# Autodesk Inventor assembly: slide with inserts
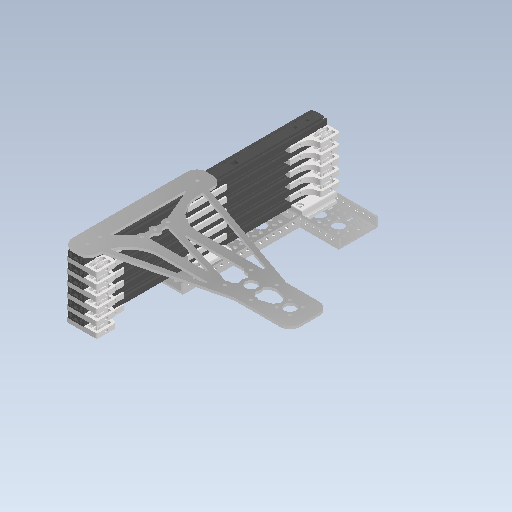
[picture p0: Inventor's stored thumbnail of the model, 512x512]
Saved by Autodesk Inventor 2020 (Build 240168000, 168)
## iProperties
Created: 2019-12-18
Part Number: slide with inserts
Document SubType Name: Assembly
Designer: xj82b
Author: xj82b
## Documents named in this file (9)
- C:\Users\xj82b\Documents\Inventor\5199\slide with inserts.iam
- C:\Users\xj82b\Documents\Inventor\5199\8x20x300mm-v2.ipt
- C:\Users\xj82b\Documents\Inventor\5199\slidesmount.ipt
- C:\Users\xj82b\Documents\Inventor\5199\rightInsertbearings.iam
- C:\Users\xj82b\Documents\Inventor\5199\leftInsertbearing.iam
- C:\Users\xj82b\Documents\Inventor\5199\centershortNEW.ipt
- C:\Users\xj82b\Documents\Inventor\5199\slidescentermount.ipt
- C:\Users\xj82b\Documents\Inventor\5199\gobilda parts\1121-0005-0144.ipt
- C:\Users\xj82b\Documents\Inventor\5199\slidesthing.ipt
## Components (27 placed, 8 different names)
1. rightInsertbearings:1 [sub-assembly] — Mate:52, Flush:26, Mate:53
2. 8x20x300mm-v2:7 — Mate:52, Flush:26, Mate:53, Mate:54, Flush:27, Mate:55, Mate:56, Mate:57, Mate:58, Mate:66, Flush:31, Flush:38, Flush:39
3. leftInsertbearing:1 [sub-assembly] — Mate:54, Flush:27, Mate:55, Flush:30
4. centershortNEW:1 — Mate:56, Mate:57, Mate:58, Mate:82
5. rightInsertbearings:2 [sub-assembly]
6. 8x20x300mm-v2:8 — Flush:31, Mate:98, Flush:46, Flush:47
7. leftInsertbearing:2 [sub-assembly] — Flush:30
8. centershortNEW:2 — Mate:66
9. 8x20x300mm-v2:9 — Mate:99, Flush:48, Mate:100, Mate:101, Mate:102, Mate:103
10. leftInsertbearing:3 [sub-assembly]
11. rightInsertbearings:4 [sub-assembly]
12. 8x20x300mm-v2:10 — Mate:82, Flush:38, Flush:39
13. leftInsertbearing:4 [sub-assembly]
14. centershortNEW:4
15. rightInsertbearings:5 [sub-assembly]
16. 8x20x300mm-v2:11 — Flush:46, Flush:47
17. leftInsertbearing:5 [sub-assembly]
18. centershortNEW:5 — Mate:98
19. rightInsertbearings:6 [sub-assembly]
20. 8x20x300mm-v2:12 — Mate:110, Mate:111, Mate:112
21. leftInsertbearing:6 [sub-assembly]
22. centershortNEW:6
23. slidesmount:2 — Mate:99, Flush:48, Mate:100, Flush:49, Mate:104, Mate:105, Mate:106
24. slidescentermount:1 — Mate:101, Mate:102, Mate:103, Flush:49, Mate:107, Mate:108
25. 1121-0005-0144:1 — Mate:107, Mate:108, Mate:109
26. 1121-0005-0144:2 — Mate:104, Mate:105, Mate:106, Mate:109
27. slidesthing:1 — Mate:110, Mate:111, Mate:112
## Relationships (79: Mate 56, Flush 23)
- Mate:52: rightInsertbearings:1 ↔ 8x20x300mm-v2:7
- Flush:26: rightInsertbearings:1 ↔ 8x20x300mm-v2:7
- Mate:53: rightInsertbearings:1 ↔ 8x20x300mm-v2:7
- Mate:54: 8x20x300mm-v2:7 ↔ leftInsertbearing:1
- Flush:27: 8x20x300mm-v2:7 ↔ leftInsertbearing:1
- Mate:55: 8x20x300mm-v2:7 ↔ leftInsertbearing:1
- Mate:56: 8x20x300mm-v2:7 ↔ centershortNEW:1
- Mate:57: 8x20x300mm-v2:7 ↔ centershortNEW:1
- Mate:58: 8x20x300mm-v2:7 ↔ centershortNEW:1
- [Mate]: rightInsertbearings:2 ↔ 8x20x300mm-v2:8
- [Flush]: rightInsertbearings:2 ↔ 8x20x300mm-v2:8
- [Mate]: rightInsertbearings:2 ↔ 8x20x300mm-v2:8
- [Mate]: 8x20x300mm-v2:8 ↔ leftInsertbearing:2
- [Flush]: 8x20x300mm-v2:8 ↔ leftInsertbearing:2
- [Mate]: 8x20x300mm-v2:8 ↔ leftInsertbearing:2
- [Mate]: 8x20x300mm-v2:8 ↔ centershortNEW:2
- [Mate]: 8x20x300mm-v2:8 ↔ centershortNEW:2
- [Mate]: 8x20x300mm-v2:8 ↔ centershortNEW:2
- Mate:66: 8x20x300mm-v2:7 ↔ centershortNEW:2
- Flush:30: leftInsertbearing:1 ↔ leftInsertbearing:2
- Flush:31: 8x20x300mm-v2:7 ↔ 8x20x300mm-v2:8
- [Mate]: 8x20x300mm-v2:9 ↔ leftInsertbearing:3
- [Flush]: 8x20x300mm-v2:9 ↔ leftInsertbearing:3
- [Mate]: 8x20x300mm-v2:9 ↔ leftInsertbearing:3
- [Mate]: rightInsertbearings:4 ↔ 8x20x300mm-v2:10
- [Flush]: rightInsertbearings:4 ↔ 8x20x300mm-v2:10
- [Mate]: rightInsertbearings:4 ↔ 8x20x300mm-v2:10
- [Mate]: 8x20x300mm-v2:10 ↔ leftInsertbearing:4
- [Flush]: 8x20x300mm-v2:10 ↔ leftInsertbearing:4
- [Mate]: 8x20x300mm-v2:10 ↔ leftInsertbearing:4
- [Mate]: 8x20x300mm-v2:10 ↔ centershortNEW:4
- [Mate]: 8x20x300mm-v2:10 ↔ centershortNEW:4
- [Mate]: 8x20x300mm-v2:10 ↔ centershortNEW:4
- [Mate]: 8x20x300mm-v2:9 ↔ centershortNEW:4
- [Flush]: leftInsertbearing:3 ↔ leftInsertbearing:4
- [Flush]: 8x20x300mm-v2:9 ↔ 8x20x300mm-v2:10
- Mate:82: centershortNEW:1 ↔ 8x20x300mm-v2:10
- Flush:38: 8x20x300mm-v2:7 ↔ 8x20x300mm-v2:10
- Flush:39: 8x20x300mm-v2:7 ↔ 8x20x300mm-v2:10
- [Mate]: rightInsertbearings:5 ↔ 8x20x300mm-v2:11
- [Flush]: rightInsertbearings:5 ↔ 8x20x300mm-v2:11
- [Mate]: rightInsertbearings:5 ↔ 8x20x300mm-v2:11
- [Mate]: 8x20x300mm-v2:11 ↔ leftInsertbearing:5
- [Flush]: 8x20x300mm-v2:11 ↔ leftInsertbearing:5
- [Mate]: 8x20x300mm-v2:11 ↔ leftInsertbearing:5
- [Mate]: 8x20x300mm-v2:11 ↔ centershortNEW:5
- [Mate]: 8x20x300mm-v2:11 ↔ centershortNEW:5
- [Mate]: 8x20x300mm-v2:11 ↔ centershortNEW:5
- [Mate]: rightInsertbearings:6 ↔ 8x20x300mm-v2:12
- [Flush]: rightInsertbearings:6 ↔ 8x20x300mm-v2:12
- [Mate]: rightInsertbearings:6 ↔ 8x20x300mm-v2:12
- [Mate]: 8x20x300mm-v2:12 ↔ leftInsertbearing:6
- [Flush]: 8x20x300mm-v2:12 ↔ leftInsertbearing:6
- [Mate]: 8x20x300mm-v2:12 ↔ leftInsertbearing:6
- [Mate]: 8x20x300mm-v2:12 ↔ centershortNEW:6
- [Mate]: 8x20x300mm-v2:12 ↔ centershortNEW:6
- [Mate]: 8x20x300mm-v2:12 ↔ centershortNEW:6
- [Mate]: 8x20x300mm-v2:11 ↔ centershortNEW:6
- [Flush]: leftInsertbearing:5 ↔ leftInsertbearing:6
- [Flush]: 8x20x300mm-v2:11 ↔ 8x20x300mm-v2:12
- Mate:98: 8x20x300mm-v2:8 ↔ centershortNEW:5
- Flush:46: 8x20x300mm-v2:8 ↔ 8x20x300mm-v2:11
- Flush:47: 8x20x300mm-v2:8 ↔ 8x20x300mm-v2:11
- Mate:99: 8x20x300mm-v2:9 ↔ slidesmount:2
- Flush:48 (2.5 mm): 8x20x300mm-v2:9 ↔ slidesmount:2
- Mate:100: 8x20x300mm-v2:9 ↔ slidesmount:2
- Mate:101: 8x20x300mm-v2:9 ↔ slidescentermount:1
- Mate:102: 8x20x300mm-v2:9 ↔ slidescentermount:1
- Mate:103: 8x20x300mm-v2:9 ↔ slidescentermount:1
- Flush:49: slidesmount:2 ↔ slidescentermount:1
- Mate:104: slidesmount:2 ↔ 1121-0005-0144:2
- Mate:105: slidesmount:2 ↔ 1121-0005-0144:2
- Mate:106: slidesmount:2 ↔ 1121-0005-0144:2
- Mate:107: slidescentermount:1 ↔ 1121-0005-0144:1
- Mate:108: slidescentermount:1 ↔ 1121-0005-0144:1
- Mate:109: 1121-0005-0144:1 ↔ 1121-0005-0144:2
- Mate:110: 8x20x300mm-v2:12 ↔ slidesthing:1
- Mate:111: 8x20x300mm-v2:12 ↔ slidesthing:1
- Mate:112: 8x20x300mm-v2:12 ↔ slidesthing:1
## Named parameters: d86_d79 = 0 mm, d87_d80 = 0 mm, d88_d81 = 0 mm, d89_d82 = 0 mm, d90_d83 = 0 mm, d91_d84 = 0 mm, d92_d85 = 0 mm, d93_d77 = 0 mm, d94_d78 = 0 mm, d98_d97 = 0 mm, d100_d80 = 0 mm, d101_d81 = 0 mm, d102_d82 = 0 mm, d106_d86_d79 = 0 mm, d107_d87_d80 = 0 mm, d108_d88_d81 = 0 mm, d109_d89_d82 = 0 mm, d110_d90_d83 = 0 mm, d111_d91_d84 = 0 mm, d112_d92_d85 = 0 mm, d113_d93_d77 = 0 mm, d114_d94_d78 = 0 mm, d115_d95 = 0 mm, d116_d96 = 0 mm, d122_d97 = 0 mm, d123_d79 = 0 mm, d124_d80 = 0 mm, d125_d81 = 0 mm, d126_d82 = 0 mm, d127_d83 = 0 mm, d128_d84 = 0 mm, d129_d85 = 0 mm, d130_d86_d79 = 0 mm, d131_d87_d80 = 0 mm, d132_d88_d81 = 0 mm, d133_d89_d82 = 0 mm, d134_d90_d83 = 0 mm, d135_d91_d84 = 0 mm, d136_d92_d85 = 0 mm, d137_d93_d77 = 0 mm, d138_d94_d78 = 0 mm, d139_d95 = 0 mm, d140_d96 = 0 mm, d141_d77 = 0 mm, d142_d78 = 0 mm
